# Autodesk Inventor assembly: BoardAssembly
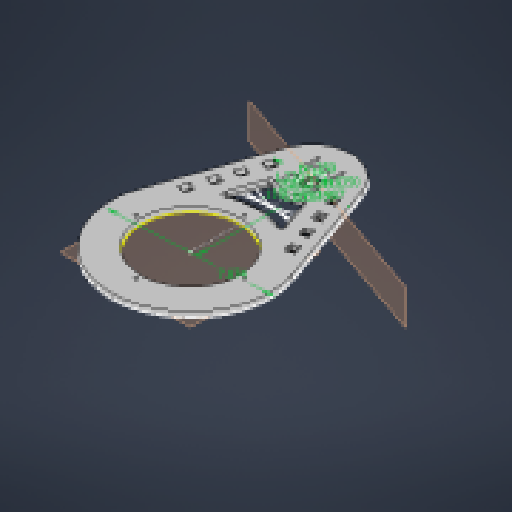
[picture p0: Inventor's stored thumbnail of the model, 512x512]
Saved by Autodesk Inventor 2024 (Build 280153000, 153)
## iProperties
Created: 2023-10-21
Part Number: BoardAssembly
Document SubType Name: Assembly
Designer: range
Author: range
## Documents named in this file (3)
- C:\Users\range\CodingProjects\C-AAM\CAD\V1\BoardAssembly.iam
- C:\Users\range\CodingProjects\C-AAM\CAD\V1\Parts\Board.ipt
- C:\Users\range\CodingProjects\C-AAM\CAD\V1\Parts\StepperBoard.ipt
## Components (2 placed, 2 different names)
1. Board:1 — Flush:1, Flush:2
2. StepperBoard:1 — Flush:1, Flush:2
## Relationships (2: Flush 2)
- Flush:1: Board:1 ↔ StepperBoard:1
- Flush:2: Board:1 ↔ StepperBoard:1
